# Autodesk Inventor assembly: stability assemb
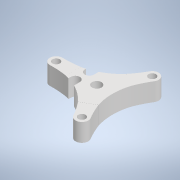
[picture p0: Inventor's stored thumbnail of the model, 180x180]
Saved by Autodesk Inventor 2020 (Build 240168000, 168)
## iProperties
Created: 2019-07-17
Part Number: stability assemb
Document SubType Name: Assembly
Designer: ColinP
Author: ColinP
## Documents named in this file (3)
- C:\Users\ColinP\Documents\Inventor\igor\stability assemb.iam
- C:\Users\ColinP\Documents\Inventor\igor\stability.ipt
- C:\Users\ColinP\Documents\Inventor\igor\screw in stablity.ipt
## Components (4 placed, 2 different names)
1. stability:1 — Insert:1, Insert:2, Insert:3, Mate:1, Mate:2, Mate:3, Mate:4
2. screw in stablity:1 — Insert:3, Mate:1
3. screw in stablity:2 — Insert:2, Mate:2
4. screw in stablity:3 — Insert:1, Mate:3, Mate:4
## Relationships (7: Mate 4, Insert 3)
- Insert:1: stability:1 ↔ screw in stablity:3
- Insert:2: stability:1 ↔ screw in stablity:2
- Insert:3: stability:1 ↔ screw in stablity:1
- Mate:1: stability:1 ↔ screw in stablity:1
- Mate:2: stability:1 ↔ screw in stablity:2
- Mate:3: stability:1 ↔ screw in stablity:3
- Mate:4: stability:1 ↔ screw in stablity:3
